# Autodesk Inventor assembly: Grundplatte_test
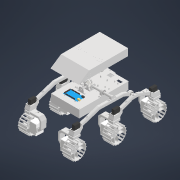
[picture p0: Inventor's stored thumbnail of the model, 180x180]
Saved by Autodesk Inventor 2021 (Build 250183000, 183)
## iProperties
Created: 2021-01-26
Part Number: Grundplatte_test
Document SubType Name: Assembly
Designer: Ctroi
Author: Ctroi
## Documents named in this file (39)
- E:\Projects\Rover\Grundplatte_test.iam
- E:\Projects\Rover\Grundplatte_hinten.ipt
- E:\Projects\Rover\Grundplatte_vorne.ipt
- E:\Projects\Rover\ArduinoMega.ipt
- E:\Projects\Rover\Kreuz_Halterung.ipt
- E:\Projects\Rover\Obenplatte_hinten.ipt
- E:\Projects\Rover\Obenplatte_vorne.ipt
- E:\Projects\Rover\Halterung_Differential_3.ipt
- E:\Projects\Rover\Halterung_Differential_Mitte.ipt
- E:\Projects\Rover\Halterung_Differential.ipt
- E:\Projects\Rover\Halterung_Differential_2.ipt
- E:\Projects\Rover\Kugellager.ipt
- E:\Projects\Rover\Kugellager_klein.ipt
- E:\Projects\Rover\Verbindung_Rocker_Body.ipt
- E:\Projects\Rover\Welle_Kugellager_Mitte.ipt
- E:\Projects\Rover\Rocker_hinten_rechts.ipt
- E:\Projects\Rover\Rocker_hinten.ipt
- E:\Projects\Rover\Rocker_vorne.ipt
- E:\Projects\Rover\Bogie.ipt
- E:\Projects\Rover\Boogie_Stange.ipt
- E:\Projects\Rover\Servohalterung_v2.ipt
- E:\Projects\Rover\Servo.ipt
- E:\Projects\Rover\Gegenstück_Welle_Diff.ipt
- E:\Projects\Rover\Zahnrad_innen.ipt
- E:\Projects\Rover\Übersetzungsbox_2.ipt
- E:\Projects\Rover\Zahnrad_außen.ipt
- E:\Projects\Rover\Motor_Servo_Welle_Test.ipt
- E:\Projects\Rover\Verbindung_Motor_Servo_v2.ipt
- E:\Projects\Rover\Motorhalterung_Klemme.ipt
- E:\Projects\Rover\Motorhalterung_v2.ipt
- E:\Projects\Rover\Steppermotor.ipt
- E:\Projects\Rover\Reifen_v2.ipt
- E:\Projects\Rover\Kegelrad.ipt
- E:\Projects\Rover\Relais.ipt
- E:\Projects\Rover\Kabelhalterung.ipt
- E:\Projects\Rover\Ebene3_vorne.ipt
- E:\Projects\Rover\Ebene3_mitte_vorne.ipt
- E:\Projects\Rover\Ebene3_hinten.ipt
- E:\Projects\Rover\Ebene3_verbindung.ipt
## Components (123 placed, 37 different names)
1. Relais:1 — Passend:208, Passend:209, Passend:210
2. Relais:2 — Passend:211, Passend:212, Passend:213
3. ArduinoMega:2 — Passend:228, Passend:229, Passend:230
4. Kabelhalterung:1 — Passend:234, Passend:235, Passend:236
5. Kabelhalterung:2 — Passend:237, Passend:238, Passend:239
6. Kabelhalterung:3 — Passend:231, Passend:232, Passend:233
7. Kabelhalterung:4 — Passend:240, Passend:241, Passend:242
8. Ebene3_vorne:1 — Passend:243, Passend:244, Passend:245, Passend:249, Passend:251
9. Ebene3_mitte_vorne:1 — Passend:246, Passend:247, Passend:248, Passend:250, Passend:252, Passend:253, Passend:254, Passend:255, Passend:256, Passend:257
10. Ebene3_hinten:1 — Passend:258, Passend:259, Passend:260
11. Ebene3_verbindung:1 — Passend:249, Passend:250, Passend:251
12. Ebene3_verbindung:2 — Passend:243, Passend:244, Passend:245, Passend:246, Passend:247, Passend:248
13. Ebene3_verbindung:3 — Passend:252, Passend:253, Passend:254
14. Ebene3_verbindung:4 — Passend:255, Passend:256, Passend:257, Passend:258, Passend:259, Passend:260
15. Grundplatte_hinten:1 — Passend:1, Passend:2, Passend:5, Passend:6, Passend:7, Passend:11, Passend:12, Passend:13, Passend:16, Passend:208, Passend:209, Passend:210, Passend:211, Passend:212, Passend:213
16. Grundplatte_vorne:1 — Passend:1, Passend:2, Passend:8, Passend:9, Passend:10, Passend:16, Passend:205, Passend:206, Passend:207
17. ArduinoMega:1 — Passend:205, Passend:206, Passend:207
18. Kreuz_Halterung:1 — Passend:5, Passend:6, Passend:7
19. Kegelrad2:1 — Passend:194, Passend:195
20. Kegelrad2:2 — Passend:196, Passend:197
21. Kegelrad2:3 — Passend:203, Passend:204
22. Gegenstück_Welle_Diff:1 — Passend:96, Passend:97
23. Welle_Kugellager_Mitte:1 — Passend:48, Passend:49, Passend:96, Passend:97, Passend:201, Passend:203, Passend:204
24. Obenplatte_vorne:1 — Passend:8, Passend:9, Passend:10, Passend:214, Passend:215, Passend:216, Passend:217, Passend:220, Passend:223, Passend:224, Passend:226, Passend:227, Passend:228, Passend:229, Passend:230, Passend:237, Passend:238, Passend:239, Passend:240, Passend:241, Passend:242
25. Halterung_Differential_3:1 — Passend:38, Passend:39, Passend:225, Passend:226, Passend:227
26. Halterung_Differential_3:2 — Passend:32, Passend:33, Passend:222, Passend:223, Passend:224
27. Obenplatte_hinten:1 — Passend:11, Passend:12, Passend:13, Passend:218, Passend:219, Passend:221, Passend:222, Passend:225, Passend:231, Passend:232, Passend:233, Passend:234, Passend:235, Passend:236
28. Halterung_Differential_Mitte:1 — Passend:42, Passend:43, Passend:214, Passend:215, Passend:216
29. Halterung_Differential:1 — Passend:36, Passend:37, Passend:199, Passend:200, Passend:217, Passend:218, Passend:219
30. Halterung_Differential:2 — Passend:34, Passend:35, Passend:198, Passend:220, Passend:221
31. Halterung_Differential_2:1 — Passend:198, Passend:199, Passend:200, Passend:201, Passend:202
32. Kugellager:1 — Passend:48, Passend:49, Passend:202
33. Kugellager:2 — Passend:32, Passend:33, Passend:47
34. Kugellager:3 — Passend:34, Passend:35, Passend:44
35. Kugellager:4 — Passend:36, Passend:37, Passend:45
36. Kugellager:5 — Passend:38, Passend:39, Passend:46
37. Kugellager_klein:1 — Passend:42, Passend:43
38. Reifen_v2:6 — Einfügen:3
39. Reifen_v2:5 — Einfügen:4
40. Reifen_v2:4 — Einfügen:5
41. Steppermotor:6 — Passend:191, Passend:192, Passend:193, Einfügen:5
42. Steppermotor:5 — Passend:188, Passend:189, Passend:190, Einfügen:4
43. Steppermotor:4 — Passend:185, Passend:186, Passend:187, Einfügen:3
44. Motorhalterung_v2:3 — Fluchtend:41, Fluchtend:42, Passend:170, Passend:185, Passend:186, Passend:187
45. Motorhalterung_v2:2 — Fluchtend:43, Fluchtend:44, Passend:171, Passend:188, Passend:189, Passend:190
46. Motorhalterung_v2:1 — Fluchtend:45, Fluchtend:46, Passend:172, Passend:191, Passend:192, Passend:193
47. Motorhalterung_Klemme:3 — Fluchtend:33, Fluchtend:34, Passend:166, Fluchtend:45, Fluchtend:46, Passend:172
48. Motorhalterung_Klemme:2 — Fluchtend:31, Fluchtend:32, Passend:165, Fluchtend:43, Fluchtend:44, Passend:171
49. Motorhalterung_Klemme:1 — Fluchtend:29, Fluchtend:30, Passend:164, Fluchtend:41, Fluchtend:42, Passend:170
50. Verbindung_Motor_Servo_v2:6 — Passend:158, Passend:159, Fluchtend:29, Fluchtend:30, Passend:164
51. Verbindung_Motor_Servo_v2:5 — Passend:162, Passend:163, Fluchtend:33, Fluchtend:34, Passend:166
52. Verbindung_Motor_Servo_v2:4 — Passend:160, Passend:161, Fluchtend:31, Fluchtend:32, Passend:165
53. Motor_Servo_Welle_Test:6 — Passend:150, Passend:151, Passend:158, Passend:159
54. Motor_Servo_Welle_Test:5 — Passend:148, Passend:149, Passend:162, Passend:163
55. Motor_Servo_Welle_Test:4 — Passend:146, Passend:147, Passend:160, Passend:161
56. Zahnrad_außen:6 — Passend:136, Passend:137
57. Zahnrad_außen:5 — Passend:138, Passend:139
58. Zahnrad_außen:4 — Passend:134, Passend:135
59. Kugellager:14 — Passend:122, Passend:123, Passend:148, Passend:149
60. Kugellager:13 — Passend:124, Passend:125, Passend:146, Passend:147
61. Kugellager:10 — Passend:126, Passend:127, Passend:150, Passend:151
62. Übersetzungsbox_2:6 — Fluchtend:25, Fluchtend:26, Passend:114, Passend:124, Passend:125
63. Übersetzungsbox_2:3 — Fluchtend:27, Fluchtend:28, Passend:115, Passend:122, Passend:123
64. Übersetzungsbox_2:2 — Fluchtend:19, Fluchtend:20, Passend:111, Passend:126, Passend:127
65. Zahnrad_innen:3 — Passend:102, Passend:103, Passend:136, Passend:137
66. Zahnrad_innen:2 — Passend:100, Passend:101, Passend:138, Passend:139
67. Zahnrad_innen:1 — Passend:98, Passend:99, Passend:134, Passend:135
68. Servo:3 — Passend:81, Passend:82, Passend:83, Passend:102, Passend:103
69. Servo:5 — Passend:93, Passend:94, Passend:95, Passend:100, Passend:101
70. Servo:2 — Passend:90, Passend:91, Passend:92, Passend:98, Passend:99
71. Servohalterung_v2:5 — Fluchtend:15, Fluchtend:16, Passend:77, Passend:90, Passend:91, Passend:92, Fluchtend:19, Fluchtend:20, Passend:111
72. Servohalterung_v2:3 — Fluchtend:13, Fluchtend:14, Passend:76, Passend:93, Passend:94, Passend:95, Fluchtend:25, Fluchtend:26, Passend:114
73. Servohalterung_v2:2 — Fluchtend:11, Fluchtend:12, Passend:75, Passend:81, Passend:82, Passend:83, Fluchtend:27, Fluchtend:28, Passend:115
74. Boogie_Stange:1 — Passend:64, Passend:65, Passend:68, Passend:69
75. Fahrwerk_bogie:2 — Passend:68, Passend:69, Fluchtend:13, Fluchtend:14, Passend:76, Fluchtend:15, Fluchtend:16, Passend:77
76. Fahrwerk_rocker_vorne:1 — Fluchtend:1, Fluchtend:2, Passend:62, Fluchtend:11, Fluchtend:12, Passend:75
77. Kugellager:7 — Passend:54, Passend:55, Passend:64, Passend:65
78. Kugellager:6 — Passend:52, Passend:53
79. Fahrwerk_rocker_hinten:1 — Passend:50, Passend:51, Passend:52, Passend:53, Passend:54, Passend:55, Fluchtend:1, Fluchtend:2, Passend:62
80. Verbindung_Rocker_Body:1 — Passend:44, Passend:47, Passend:50, Passend:51, Passend:194, Passend:195
81. Reifen_v2:3 — Einfügen:2
82. Reifen_v2:2 — Einfügen:1
83. Reifen_v2:1 — Einfügen:6
84. Steppermotor:3 — Passend:182, Passend:183, Passend:184, Einfügen:6
85. Steppermotor:2 — Passend:179, Passend:180, Passend:181, Einfügen:2
86. Steppermotor:1 — Passend:176, Passend:177, Passend:178, Einfügen:1
87. Motorhalterung_v2:6 — Fluchtend:51, Fluchtend:52, Passend:175, Passend:182, Passend:183, Passend:184
88. Motorhalterung_v2:5 — Fluchtend:49, Fluchtend:50, Passend:174, Passend:179, Passend:180, Passend:181
89. Motorhalterung_v2:4 — Fluchtend:47, Fluchtend:48, Passend:173, Passend:176, Passend:177, Passend:178
90. Motorhalterung_Klemme:4 — Fluchtend:35, Fluchtend:36, Passend:167, Fluchtend:47, Fluchtend:48, Passend:173
91. Motorhalterung_Klemme:5 — Fluchtend:37, Fluchtend:38, Passend:168, Fluchtend:49, Fluchtend:50, Passend:174
92. Motorhalterung_Klemme:6 — Fluchtend:39, Fluchtend:40, Passend:169, Fluchtend:51, Fluchtend:52, Passend:175
93. Verbindung_Motor_Servo_v2:3 — Passend:152, Passend:153, Fluchtend:35, Fluchtend:36, Passend:167
94. Verbindung_Motor_Servo_v2:2 — Passend:156, Passend:157, Fluchtend:39, Fluchtend:40, Passend:169
95. Verbindung_Motor_Servo_v2:1 — Passend:154, Passend:155, Fluchtend:37, Fluchtend:38, Passend:168
96. Motor_Servo_Welle_Test:3 — Passend:144, Passend:145, Passend:156, Passend:157
97. Motor_Servo_Welle_Test:2 — Passend:140, Passend:141, Passend:152, Passend:153
98. Motor_Servo_Welle_Test:1 — Passend:142, Passend:143, Passend:154, Passend:155
99. Zahnrad_außen:3 — Passend:132, Passend:133
100. Zahnrad_außen:2 — Passend:130, Passend:131
101. Zahnrad_außen:1 — Passend:128, Passend:129
102. Kugellager:15 — Passend:120, Passend:121, Passend:140, Passend:141
103. Kugellager:12 — Passend:118, Passend:119, Passend:142, Passend:143
104. Kugellager:11 — Passend:116, Passend:117, Passend:144, Passend:145
105. Übersetzungsbox_2:5 — Fluchtend:21, Fluchtend:22, Passend:112, Passend:118, Passend:119
106. Übersetzungsbox_2:4 — Fluchtend:23, Fluchtend:24, Passend:113, Passend:120, Passend:121
107. Übersetzungsbox_2:1 — Fluchtend:17, Fluchtend:18, Passend:110, Passend:116, Passend:117
108. Zahnrad_innen:6 — Passend:108, Passend:109, Passend:132, Passend:133
109. Zahnrad_innen:5 — Passend:106, Passend:107, Passend:130, Passend:131
110. Zahnrad_innen:4 — Passend:104, Passend:105, Passend:128, Passend:129
111. Servo:4 — Passend:78, Passend:79, Passend:80, Passend:108, Passend:109
112. Servo:6 — Passend:84, Passend:85, Passend:86, Passend:106, Passend:107
113. Servo:1 — Passend:87, Passend:88, Passend:89, Passend:104, Passend:105
114. Servohalterung_v2:6 — Fluchtend:5, Fluchtend:6, Passend:72, Passend:87, Passend:88, Passend:89, Fluchtend:17, Fluchtend:18, Passend:110
115. Servohalterung_v2:4 — Fluchtend:7, Fluchtend:8, Passend:73, Passend:84, Passend:85, Passend:86, Fluchtend:21, Fluchtend:22, Passend:112
116. Servohalterung_v2:1 — Fluchtend:9, Fluchtend:10, Passend:74, Passend:78, Passend:79, Passend:80, Fluchtend:23, Fluchtend:24, Passend:113
117. Boogie_Stange:2 — Passend:66, Passend:67, Passend:70, Passend:71
118. Fahrwerk_bogie:1 — Passend:70, Passend:71, Fluchtend:5, Fluchtend:6, Passend:72, Fluchtend:7, Fluchtend:8, Passend:73
119. Kugellager:9 — Passend:60, Passend:61
120. Kugellager:8 — Passend:58, Passend:59, Passend:66, Passend:67
121. Fahrwerk_rocker_hinten:2 — Passend:56, Passend:57, Passend:58, Passend:59, Passend:60, Passend:61, Fluchtend:3, Fluchtend:4, Passend:63
122. Fahrwerk_rocker_vorne:2 — Fluchtend:3, Fluchtend:4, Passend:63, Fluchtend:9, Fluchtend:10, Passend:74
123. Verbindung_Rocker_Body:2 — Passend:45, Passend:46, Passend:56, Passend:57, Passend:196, Passend:197
## Relationships (297: Mate 239, Flush 52, Insert 6)
- Passend:1 [Mate]: Grundplatte_hinten:1 ↔ Grundplatte_vorne:1
- Passend:2 [Mate]: Grundplatte_hinten:1 ↔ Grundplatte_vorne:1
- Passend:5 [Mate]: Grundplatte_hinten:1 ↔ Kreuz_Halterung:1
- Passend:6 [Mate]: Grundplatte_hinten:1 ↔ Kreuz_Halterung:1
- Passend:7 [Mate]: Grundplatte_hinten:1 ↔ Kreuz_Halterung:1
- Passend:8 [Mate]: Grundplatte_vorne:1 ↔ Obenplatte_vorne:1
- Passend:9 [Mate]: Grundplatte_vorne:1 ↔ Obenplatte_vorne:1
- Passend:10 [Mate]: Grundplatte_vorne:1 ↔ Obenplatte_vorne:1
- Passend:11 [Mate]: Grundplatte_hinten:1 ↔ Obenplatte_hinten:1
- Passend:12 [Mate]: Grundplatte_hinten:1 ↔ Obenplatte_hinten:1
- Passend:13 [Mate]: Grundplatte_hinten:1 ↔ Obenplatte_hinten:1
- Passend:16 [Mate]: Grundplatte_hinten:1 ↔ Grundplatte_vorne:1
- Passend:32 [Mate]: Halterung_Differential_3:2 ↔ Kugellager:2
- Passend:33 [Mate]: Halterung_Differential_3:2 ↔ Kugellager:2
- Passend:34 [Mate]: Halterung_Differential:2 ↔ Kugellager:3
- Passend:35 [Mate]: Halterung_Differential:2 ↔ Kugellager:3
- Passend:36 [Mate]: Halterung_Differential:1 ↔ Kugellager:4
- Passend:37 [Mate]: Halterung_Differential:1 ↔ Kugellager:4
- Passend:38 [Mate]: Halterung_Differential_3:1 ↔ Kugellager:5
- Passend:39 [Mate]: Halterung_Differential_3:1 ↔ Kugellager:5
- Passend:42 [Mate]: Halterung_Differential_Mitte:1 ↔ Kugellager_klein:1
- Passend:43 [Mate]: Halterung_Differential_Mitte:1 ↔ Kugellager_klein:1
- Passend:44 [Mate]: Kugellager:3 ↔ Verbindung_Rocker_Body:1
- Passend:45 [Mate]: Kugellager:4 ↔ Verbindung_Rocker_Body:2
- Passend:46 [Mate]: Kugellager:5 ↔ Verbindung_Rocker_Body:2
- Passend:47 [Mate]: Kugellager:2 ↔ Verbindung_Rocker_Body:1
- Passend:48 [Mate]: Welle_Kugellager_Mitte:1 ↔ Kugellager:1
- Passend:49 [Mate]: Welle_Kugellager_Mitte:1 ↔ Kugellager:1
- Passend:50 [Mate]: Fahrwerk_rocker_hinten:1 ↔ Verbindung_Rocker_Body:1
- Passend:51 [Mate]: Fahrwerk_rocker_hinten:1 ↔ Verbindung_Rocker_Body:1
- Passend:52 [Mate]: Kugellager:6 ↔ Fahrwerk_rocker_hinten:1
- Passend:53 [Mate]: Kugellager:6 ↔ Fahrwerk_rocker_hinten:1
- Passend:54 [Mate]: Kugellager:7 ↔ Fahrwerk_rocker_hinten:1
- Passend:55 [Mate]: Kugellager:7 ↔ Fahrwerk_rocker_hinten:1
- Passend:56 [Mate]: Fahrwerk_rocker_hinten:2 ↔ Verbindung_Rocker_Body:2
- Passend:57 [Mate]: Fahrwerk_rocker_hinten:2 ↔ Verbindung_Rocker_Body:2
- Passend:58 [Mate]: Kugellager:8 ↔ Fahrwerk_rocker_hinten:2
- Passend:59 [Mate]: Kugellager:8 ↔ Fahrwerk_rocker_hinten:2
- Passend:60 [Mate]: Kugellager:9 ↔ Fahrwerk_rocker_hinten:2
- Passend:61 [Mate]: Kugellager:9 ↔ Fahrwerk_rocker_hinten:2
- Fluchtend:1 [Flush]: Fahrwerk_rocker_vorne:1 ↔ Fahrwerk_rocker_hinten:1
- Fluchtend:2 [Flush]: Fahrwerk_rocker_vorne:1 ↔ Fahrwerk_rocker_hinten:1
- Passend:62 [Mate]: Fahrwerk_rocker_vorne:1 ↔ Fahrwerk_rocker_hinten:1
- Fluchtend:3 [Flush]: Fahrwerk_rocker_hinten:2 ↔ Fahrwerk_rocker_vorne:2
- Fluchtend:4 [Flush]: Fahrwerk_rocker_hinten:2 ↔ Fahrwerk_rocker_vorne:2
- Passend:63 [Mate]: Fahrwerk_rocker_hinten:2 ↔ Fahrwerk_rocker_vorne:2
- Passend:64 [Mate]: Boogie_Stange:1 ↔ Kugellager:7
- Passend:65 [Mate]: Boogie_Stange:1 ↔ Kugellager:7
- Passend:66 [Mate]: Boogie_Stange:2 ↔ Kugellager:8
- Passend:67 [Mate]: Boogie_Stange:2 ↔ Kugellager:8
- Passend:68 [Mate]: Boogie_Stange:1 ↔ Fahrwerk_bogie:2
- Passend:69 [Mate]: Boogie_Stange:1 ↔ Fahrwerk_bogie:2
- Passend:70 [Mate]: Boogie_Stange:2 ↔ Fahrwerk_bogie:1
- Passend:71 [Mate]: Boogie_Stange:2 ↔ Fahrwerk_bogie:1
- Fluchtend:5 [Flush]: Servohalterung_v2:6 ↔ Fahrwerk_bogie:1
- Fluchtend:6 [Flush]: Servohalterung_v2:6 ↔ Fahrwerk_bogie:1
- Passend:72 [Mate]: Servohalterung_v2:6 ↔ Fahrwerk_bogie:1
- Fluchtend:7 [Flush]: Servohalterung_v2:4 ↔ Fahrwerk_bogie:1
- Fluchtend:8 [Flush]: Servohalterung_v2:4 ↔ Fahrwerk_bogie:1
- Passend:73 [Mate]: Servohalterung_v2:4 ↔ Fahrwerk_bogie:1
- Fluchtend:9 [Flush]: Servohalterung_v2:1 ↔ Fahrwerk_rocker_vorne:2
- Fluchtend:10 [Flush]: Servohalterung_v2:1 ↔ Fahrwerk_rocker_vorne:2
- Passend:74 [Mate]: Servohalterung_v2:1 ↔ Fahrwerk_rocker_vorne:2
- Fluchtend:11 [Flush]: Servohalterung_v2:2 ↔ Fahrwerk_rocker_vorne:1
- Fluchtend:12 [Flush]: Servohalterung_v2:2 ↔ Fahrwerk_rocker_vorne:1
- Passend:75 [Mate]: Servohalterung_v2:2 ↔ Fahrwerk_rocker_vorne:1
- Fluchtend:13 [Flush]: Servohalterung_v2:3 ↔ Fahrwerk_bogie:2
- Fluchtend:14 [Flush]: Servohalterung_v2:3 ↔ Fahrwerk_bogie:2
- Passend:76 [Mate]: Servohalterung_v2:3 ↔ Fahrwerk_bogie:2
- Fluchtend:15 [Flush]: Servohalterung_v2:5 ↔ Fahrwerk_bogie:2
- Fluchtend:16 [Flush]: Servohalterung_v2:5 ↔ Fahrwerk_bogie:2
- Passend:77 [Mate]: Servohalterung_v2:5 ↔ Fahrwerk_bogie:2
- Passend:78 [Mate]: Servo:4 ↔ Servohalterung_v2:1
- Passend:79 [Mate]: Servo:4 ↔ Servohalterung_v2:1
- Passend:80 [Mate]: Servo:4 ↔ Servohalterung_v2:1
- Passend:81 [Mate]: Servo:3 ↔ Servohalterung_v2:2
- Passend:82 [Mate]: Servo:3 ↔ Servohalterung_v2:2
- Passend:83 [Mate]: Servo:3 ↔ Servohalterung_v2:2
- Passend:84 [Mate]: Servo:6 ↔ Servohalterung_v2:4
- Passend:85 [Mate]: Servo:6 ↔ Servohalterung_v2:4
- Passend:86 [Mate]: Servo:6 ↔ Servohalterung_v2:4
- Passend:87 [Mate]: Servo:1 ↔ Servohalterung_v2:6
- Passend:88 [Mate]: Servo:1 ↔ Servohalterung_v2:6
- Passend:89 [Mate]: Servo:1 ↔ Servohalterung_v2:6
- Passend:90 [Mate]: Servo:2 ↔ Servohalterung_v2:5
- Passend:91 [Mate]: Servo:2 ↔ Servohalterung_v2:5
- Passend:92 [Mate]: Servo:2 ↔ Servohalterung_v2:5
- Passend:93 [Mate]: Servo:5 ↔ Servohalterung_v2:3
- Passend:94 [Mate]: Servo:5 ↔ Servohalterung_v2:3
- Passend:95 [Mate]: Servo:5 ↔ Servohalterung_v2:3
- Passend:96 [Mate]: Gegenstück_Welle_Diff:1 ↔ Welle_Kugellager_Mitte:1
- Passend:97 [Mate]: Gegenstück_Welle_Diff:1 ↔ Welle_Kugellager_Mitte:1
- Passend:98 [Mate]: Zahnrad_innen:1 ↔ Servo:2
- Passend:99 [Mate]: Zahnrad_innen:1 ↔ Servo:2
- Passend:100 [Mate]: Zahnrad_innen:2 ↔ Servo:5
- Passend:101 [Mate]: Zahnrad_innen:2 ↔ Servo:5
- Passend:102 [Mate]: Zahnrad_innen:3 ↔ Servo:3
- Passend:103 [Mate]: Zahnrad_innen:3 ↔ Servo:3
- Passend:104 [Mate]: Zahnrad_innen:4 ↔ Servo:1
- Passend:105 [Mate]: Zahnrad_innen:4 ↔ Servo:1
- Passend:106 [Mate]: Zahnrad_innen:5 ↔ Servo:6
- Passend:107 [Mate]: Zahnrad_innen:5 ↔ Servo:6
- Passend:108 [Mate]: Zahnrad_innen:6 ↔ Servo:4
- Passend:109 [Mate]: Zahnrad_innen:6 ↔ Servo:4
- Fluchtend:17 [Flush]: Übersetzungsbox_2:1 ↔ Servohalterung_v2:6
- Fluchtend:18 [Flush]: Übersetzungsbox_2:1 ↔ Servohalterung_v2:6
- Passend:110 [Mate]: Übersetzungsbox_2:1 ↔ Servohalterung_v2:6
- Fluchtend:19 [Flush]: Übersetzungsbox_2:2 ↔ Servohalterung_v2:5
- Fluchtend:20 [Flush]: Übersetzungsbox_2:2 ↔ Servohalterung_v2:5
- Passend:111 [Mate]: Übersetzungsbox_2:2 ↔ Servohalterung_v2:5
- Fluchtend:21 [Flush]: Übersetzungsbox_2:5 ↔ Servohalterung_v2:4
- Fluchtend:22 [Flush]: Übersetzungsbox_2:5 ↔ Servohalterung_v2:4
- Passend:112 [Mate]: Übersetzungsbox_2:5 ↔ Servohalterung_v2:4
- Fluchtend:23 [Flush]: Übersetzungsbox_2:4 ↔ Servohalterung_v2:1
- Fluchtend:24 [Flush]: Übersetzungsbox_2:4 ↔ Servohalterung_v2:1
- Passend:113 [Mate]: Übersetzungsbox_2:4 ↔ Servohalterung_v2:1
- Fluchtend:25 [Flush]: Übersetzungsbox_2:6 ↔ Servohalterung_v2:3
- Fluchtend:26 [Flush]: Übersetzungsbox_2:6 ↔ Servohalterung_v2:3
- Passend:114 [Mate]: Übersetzungsbox_2:6 ↔ Servohalterung_v2:3
- Fluchtend:27 [Flush]: Übersetzungsbox_2:3 ↔ Servohalterung_v2:2
- Fluchtend:28 [Flush]: Übersetzungsbox_2:3 ↔ Servohalterung_v2:2
- Passend:115 [Mate]: Übersetzungsbox_2:3 ↔ Servohalterung_v2:2
- Passend:116 [Mate]: Kugellager:11 ↔ Übersetzungsbox_2:1
- Passend:117 [Mate]: Kugellager:11 ↔ Übersetzungsbox_2:1
- Passend:118 [Mate]: Kugellager:12 ↔ Übersetzungsbox_2:5
- Passend:119 [Mate]: Kugellager:12 ↔ Übersetzungsbox_2:5
- Passend:120 [Mate]: Kugellager:15 ↔ Übersetzungsbox_2:4
- Passend:121 [Mate]: Kugellager:15 ↔ Übersetzungsbox_2:4
- Passend:122 [Mate]: Kugellager:14 ↔ Übersetzungsbox_2:3
- Passend:123 [Mate]: Kugellager:14 ↔ Übersetzungsbox_2:3
- Passend:124 [Mate]: Kugellager:13 ↔ Übersetzungsbox_2:6
- Passend:125 [Mate]: Kugellager:13 ↔ Übersetzungsbox_2:6
- Passend:126 [Mate]: Kugellager:10 ↔ Übersetzungsbox_2:2
- Passend:127 [Mate]: Kugellager:10 ↔ Übersetzungsbox_2:2
- Passend:128 [Mate]: Zahnrad_außen:1 ↔ Zahnrad_innen:4
- Passend:129 [Mate]: Zahnrad_außen:1 ↔ Zahnrad_innen:4
- Passend:130 [Mate]: Zahnrad_außen:2 ↔ Zahnrad_innen:5
- Passend:131 [Mate]: Zahnrad_außen:2 ↔ Zahnrad_innen:5
- Passend:132 [Mate]: Zahnrad_außen:3 ↔ Zahnrad_innen:6
- Passend:133 [Mate]: Zahnrad_außen:3 ↔ Zahnrad_innen:6
- Passend:134 [Mate]: Zahnrad_außen:4 ↔ Zahnrad_innen:1
- Passend:135 [Mate]: Zahnrad_außen:4 ↔ Zahnrad_innen:1
- Passend:136 [Mate]: Zahnrad_außen:6 ↔ Zahnrad_innen:3
- Passend:137 [Mate]: Zahnrad_außen:6 ↔ Zahnrad_innen:3
- Passend:138 [Mate]: Zahnrad_außen:5 ↔ Zahnrad_innen:2
- Passend:139 [Mate]: Zahnrad_außen:5 ↔ Zahnrad_innen:2
- Passend:140 [Mate]: Motor_Servo_Welle_Test:2 ↔ Kugellager:15
- Passend:141 [Mate]: Motor_Servo_Welle_Test:2 ↔ Kugellager:15
- Passend:142 [Mate]: Motor_Servo_Welle_Test:1 ↔ Kugellager:12
- Passend:143 [Mate]: Motor_Servo_Welle_Test:1 ↔ Kugellager:12
- Passend:144 [Mate]: Motor_Servo_Welle_Test:3 ↔ Kugellager:11
- Passend:145 [Mate]: Motor_Servo_Welle_Test:3 ↔ Kugellager:11
- Passend:146 [Mate]: Motor_Servo_Welle_Test:4 ↔ Kugellager:13
- Passend:147 [Mate]: Motor_Servo_Welle_Test:4 ↔ Kugellager:13
- Passend:148 [Mate]: Motor_Servo_Welle_Test:5 ↔ Kugellager:14
- Passend:149 [Mate]: Motor_Servo_Welle_Test:5 ↔ Kugellager:14
- Passend:150 [Mate]: Motor_Servo_Welle_Test:6 ↔ Kugellager:10
- Passend:151 [Mate]: Motor_Servo_Welle_Test:6 ↔ Kugellager:10
- Passend:152 [Mate]: Verbindung_Motor_Servo_v2:3 ↔ Motor_Servo_Welle_Test:2
- Passend:153 [Mate]: Verbindung_Motor_Servo_v2:3 ↔ Motor_Servo_Welle_Test:2
- Passend:154 [Mate]: Verbindung_Motor_Servo_v2:1 ↔ Motor_Servo_Welle_Test:1
- Passend:155 [Mate]: Verbindung_Motor_Servo_v2:1 ↔ Motor_Servo_Welle_Test:1
- Passend:156 [Mate]: Verbindung_Motor_Servo_v2:2 ↔ Motor_Servo_Welle_Test:3
- Passend:157 [Mate]: Verbindung_Motor_Servo_v2:2 ↔ Motor_Servo_Welle_Test:3
- Passend:158 [Mate]: Verbindung_Motor_Servo_v2:6 ↔ Motor_Servo_Welle_Test:6
- Passend:159 [Mate]: Verbindung_Motor_Servo_v2:6 ↔ Motor_Servo_Welle_Test:6
- Passend:160 [Mate]: Verbindung_Motor_Servo_v2:4 ↔ Motor_Servo_Welle_Test:4
- Passend:161 [Mate]: Verbindung_Motor_Servo_v2:4 ↔ Motor_Servo_Welle_Test:4
- Passend:162 [Mate]: Verbindung_Motor_Servo_v2:5 ↔ Motor_Servo_Welle_Test:5
- Passend:163 [Mate]: Verbindung_Motor_Servo_v2:5 ↔ Motor_Servo_Welle_Test:5
- Fluchtend:29 [Flush]: Motorhalterung_Klemme:1 ↔ Verbindung_Motor_Servo_v2:6
- Fluchtend:30 [Flush]: Motorhalterung_Klemme:1 ↔ Verbindung_Motor_Servo_v2:6
- Passend:164 [Mate]: Motorhalterung_Klemme:1 ↔ Verbindung_Motor_Servo_v2:6
- Fluchtend:31 [Flush]: Motorhalterung_Klemme:2 ↔ Verbindung_Motor_Servo_v2:4
- Fluchtend:32 [Flush]: Motorhalterung_Klemme:2 ↔ Verbindung_Motor_Servo_v2:4
- Passend:165 [Mate]: Motorhalterung_Klemme:2 ↔ Verbindung_Motor_Servo_v2:4
- Fluchtend:33 [Flush]: Motorhalterung_Klemme:3 ↔ Verbindung_Motor_Servo_v2:5
- Fluchtend:34 [Flush]: Motorhalterung_Klemme:3 ↔ Verbindung_Motor_Servo_v2:5
- Passend:166 [Mate]: Motorhalterung_Klemme:3 ↔ Verbindung_Motor_Servo_v2:5
- Fluchtend:35 [Flush]: Motorhalterung_Klemme:4 ↔ Verbindung_Motor_Servo_v2:3
- Fluchtend:36 [Flush]: Motorhalterung_Klemme:4 ↔ Verbindung_Motor_Servo_v2:3
- Passend:167 [Mate]: Motorhalterung_Klemme:4 ↔ Verbindung_Motor_Servo_v2:3
- Fluchtend:37 [Flush]: Motorhalterung_Klemme:5 ↔ Verbindung_Motor_Servo_v2:1
- Fluchtend:38 [Flush]: Motorhalterung_Klemme:5 ↔ Verbindung_Motor_Servo_v2:1
- Passend:168 [Mate]: Motorhalterung_Klemme:5 ↔ Verbindung_Motor_Servo_v2:1
- Fluchtend:39 [Flush]: Motorhalterung_Klemme:6 ↔ Verbindung_Motor_Servo_v2:2
- Fluchtend:40 [Flush]: Motorhalterung_Klemme:6 ↔ Verbindung_Motor_Servo_v2:2
- Passend:169 [Mate]: Motorhalterung_Klemme:6 ↔ Verbindung_Motor_Servo_v2:2
- Fluchtend:41 [Flush]: Motorhalterung_v2:3 ↔ Motorhalterung_Klemme:1
- Fluchtend:42 [Flush]: Motorhalterung_v2:3 ↔ Motorhalterung_Klemme:1
- Passend:170 [Mate]: Motorhalterung_v2:3 ↔ Motorhalterung_Klemme:1
- Fluchtend:43 [Flush]: Motorhalterung_v2:2 ↔ Motorhalterung_Klemme:2
- Fluchtend:44 [Flush]: Motorhalterung_v2:2 ↔ Motorhalterung_Klemme:2
- Passend:171 [Mate]: Motorhalterung_v2:2 ↔ Motorhalterung_Klemme:2
- Fluchtend:45 [Flush]: Motorhalterung_v2:1 ↔ Motorhalterung_Klemme:3
- Fluchtend:46 [Flush]: Motorhalterung_v2:1 ↔ Motorhalterung_Klemme:3
- Passend:172 [Mate]: Motorhalterung_v2:1 ↔ Motorhalterung_Klemme:3
- Fluchtend:47 [Flush]: Motorhalterung_v2:4 ↔ Motorhalterung_Klemme:4
- Fluchtend:48 [Flush]: Motorhalterung_v2:4 ↔ Motorhalterung_Klemme:4
- Passend:173 [Mate]: Motorhalterung_v2:4 ↔ Motorhalterung_Klemme:4
- Fluchtend:49 [Flush]: Motorhalterung_v2:5 ↔ Motorhalterung_Klemme:5
- Fluchtend:50 [Flush]: Motorhalterung_v2:5 ↔ Motorhalterung_Klemme:5
- Passend:174 [Mate]: Motorhalterung_v2:5 ↔ Motorhalterung_Klemme:5
- Fluchtend:51 [Flush]: Motorhalterung_v2:6 ↔ Motorhalterung_Klemme:6
- Fluchtend:52 [Flush]: Motorhalterung_v2:6 ↔ Motorhalterung_Klemme:6
- Passend:175 [Mate]: Motorhalterung_v2:6 ↔ Motorhalterung_Klemme:6
- Passend:176 [Mate]: Steppermotor:1 ↔ Motorhalterung_v2:4
- Passend:177 [Mate]: Steppermotor:1 ↔ Motorhalterung_v2:4
- Passend:178 [Mate]: Steppermotor:1 ↔ Motorhalterung_v2:4
- Passend:179 [Mate]: Steppermotor:2 ↔ Motorhalterung_v2:5
- Passend:180 [Mate]: Steppermotor:2 ↔ Motorhalterung_v2:5
- Passend:181 [Mate]: Steppermotor:2 ↔ Motorhalterung_v2:5
- Passend:182 [Mate]: Steppermotor:3 ↔ Motorhalterung_v2:6
- Passend:183 [Mate]: Steppermotor:3 ↔ Motorhalterung_v2:6
- Passend:184 [Mate]: Steppermotor:3 ↔ Motorhalterung_v2:6
- Passend:185 [Mate]: Steppermotor:4 ↔ Motorhalterung_v2:3
- Passend:186 [Mate]: Steppermotor:4 ↔ Motorhalterung_v2:3
- Passend:187 [Mate]: Steppermotor:4 ↔ Motorhalterung_v2:3
- Passend:188 [Mate]: Steppermotor:5 ↔ Motorhalterung_v2:2
- Passend:189 [Mate]: Steppermotor:5 ↔ Motorhalterung_v2:2
- Passend:190 [Mate]: Steppermotor:5 ↔ Motorhalterung_v2:2
- Passend:191 [Mate]: Steppermotor:6 ↔ Motorhalterung_v2:1
- Passend:192 [Mate]: Steppermotor:6 ↔ Motorhalterung_v2:1
- Passend:193 [Mate]: Steppermotor:6 ↔ Motorhalterung_v2:1
- Einfügen:1 [Insert] (-15 mm): Reifen_v2:2 ↔ Steppermotor:1
- Einfügen:2 [Insert] (-15 mm): Reifen_v2:3 ↔ Steppermotor:2
- Einfügen:3 [Insert] (-15 mm): Reifen_v2:6 ↔ Steppermotor:4
- Einfügen:4 [Insert] (-15 mm): Reifen_v2:5 ↔ Steppermotor:5
- Einfügen:5 [Insert] (-15 mm): Reifen_v2:4 ↔ Steppermotor:6
- Passend:194 [Mate]: Kegelrad2:1 ↔ Verbindung_Rocker_Body:1
- Passend:195 [Mate]: Kegelrad2:1 ↔ Verbindung_Rocker_Body:1
- Passend:196 [Mate]: Kegelrad2:2 ↔ Verbindung_Rocker_Body:2
- Passend:197 [Mate]: Kegelrad2:2 ↔ Verbindung_Rocker_Body:2
- Passend:198 [Mate]: Halterung_Differential:2 ↔ Halterung_Differential_2:1
- Passend:199 [Mate]: Halterung_Differential:1 ↔ Halterung_Differential_2:1
- Passend:200 [Mate]: Halterung_Differential:1 ↔ Halterung_Differential_2:1
- Passend:201 [Mate]: Welle_Kugellager_Mitte:1 ↔ Halterung_Differential_2:1
- Passend:202 [Mate]: Halterung_Differential_2:1 ↔ Kugellager:1
- Passend:203 [Mate]: Kegelrad2:3 ↔ Welle_Kugellager_Mitte:1
- Passend:204 [Mate]: Kegelrad2:3 ↔ Welle_Kugellager_Mitte:1
- Einfügen:6 [Insert] (-15 mm): Reifen_v2:1 ↔ Steppermotor:3
- Passend:205 [Mate]: Grundplatte_vorne:1 ↔ ArduinoMega:1
- Passend:206 [Mate]: Grundplatte_vorne:1 ↔ ArduinoMega:1
- Passend:207 [Mate]: Grundplatte_vorne:1 ↔ ArduinoMega:1
- Passend:208 [Mate]: Relais:1 ↔ Grundplatte_hinten:1
- Passend:209 [Mate]: Relais:1 ↔ Grundplatte_hinten:1
- Passend:210 [Mate]: Relais:1 ↔ Grundplatte_hinten:1
- Passend:211 [Mate]: Relais:2 ↔ Grundplatte_hinten:1
- Passend:212 [Mate]: Relais:2 ↔ Grundplatte_hinten:1
- Passend:213 [Mate]: Relais:2 ↔ Grundplatte_hinten:1
- Passend:214 [Mate]: Obenplatte_vorne:1 ↔ Halterung_Differential_Mitte:1
- Passend:215 [Mate]: Obenplatte_vorne:1 ↔ Halterung_Differential_Mitte:1
- Passend:216 [Mate]: Obenplatte_vorne:1 ↔ Halterung_Differential_Mitte:1
- Passend:217 [Mate]: Obenplatte_vorne:1 ↔ Halterung_Differential:1
- Passend:218 [Mate]: Obenplatte_hinten:1 ↔ Halterung_Differential:1
- Passend:219 [Mate]: Obenplatte_hinten:1 ↔ Halterung_Differential:1
- Passend:220 [Mate]: Obenplatte_vorne:1 ↔ Halterung_Differential:2
- Passend:221 [Mate]: Obenplatte_hinten:1 ↔ Halterung_Differential:2
- Passend:222 [Mate]: Halterung_Differential_3:2 ↔ Obenplatte_hinten:1
- Passend:223 [Mate]: Obenplatte_vorne:1 ↔ Halterung_Differential_3:2
- Passend:224 [Mate]: Obenplatte_vorne:1 ↔ Halterung_Differential_3:2
- Passend:225 [Mate]: Halterung_Differential_3:1 ↔ Obenplatte_hinten:1
- Passend:226 [Mate]: Obenplatte_vorne:1 ↔ Halterung_Differential_3:1
- Passend:227 [Mate]: Obenplatte_vorne:1 ↔ Halterung_Differential_3:1
- Passend:228 [Mate]: ArduinoMega:2 ↔ Obenplatte_vorne:1
- Passend:229 [Mate]: ArduinoMega:2 ↔ Obenplatte_vorne:1
- Passend:230 [Mate]: ArduinoMega:2 ↔ Obenplatte_vorne:1
- Passend:231 [Mate]: Kabelhalterung:3 ↔ Obenplatte_hinten:1
- Passend:232 [Mate]: Kabelhalterung:3 ↔ Obenplatte_hinten:1
- Passend:233 [Mate]: Kabelhalterung:3 ↔ Obenplatte_hinten:1
- Passend:234 [Mate]: Kabelhalterung:1 ↔ Obenplatte_hinten:1
- Passend:235 [Mate]: Kabelhalterung:1 ↔ Obenplatte_hinten:1
- Passend:236 [Mate]: Kabelhalterung:1 ↔ Obenplatte_hinten:1
- Passend:237 [Mate]: Kabelhalterung:2 ↔ Obenplatte_vorne:1
- Passend:238 [Mate]: Kabelhalterung:2 ↔ Obenplatte_vorne:1
- Passend:239 [Mate]: Kabelhalterung:2 ↔ Obenplatte_vorne:1
- Passend:240 [Mate]: Kabelhalterung:4 ↔ Obenplatte_vorne:1
- Passend:241 [Mate]: Kabelhalterung:4 ↔ Obenplatte_vorne:1
- Passend:242 [Mate]: Kabelhalterung:4 ↔ Obenplatte_vorne:1
- Passend:243 [Mate]: Ebene3_vorne:1 ↔ Ebene3_verbindung:2
- Passend:244 [Mate]: Ebene3_vorne:1 ↔ Ebene3_verbindung:2
- Passend:245 [Mate]: Ebene3_vorne:1 ↔ Ebene3_verbindung:2
- Passend:246 [Mate]: Ebene3_mitte_vorne:1 ↔ Ebene3_verbindung:2
- Passend:247 [Mate]: Ebene3_mitte_vorne:1 ↔ Ebene3_verbindung:2
- Passend:248 [Mate]: Ebene3_mitte_vorne:1 ↔ Ebene3_verbindung:2
- Passend:249 [Mate]: Ebene3_vorne:1 ↔ Ebene3_verbindung:1
- Passend:250 [Mate]: Ebene3_mitte_vorne:1 ↔ Ebene3_verbindung:1
- Passend:251 [Mate]: Ebene3_vorne:1 ↔ Ebene3_verbindung:1
- Passend:252 [Mate]: Ebene3_mitte_vorne:1 ↔ Ebene3_verbindung:3
- Passend:253 [Mate]: Ebene3_mitte_vorne:1 ↔ Ebene3_verbindung:3
- Passend:254 [Mate]: Ebene3_mitte_vorne:1 ↔ Ebene3_verbindung:3
- Passend:255 [Mate]: Ebene3_mitte_vorne:1 ↔ Ebene3_verbindung:4
- Passend:256 [Mate]: Ebene3_mitte_vorne:1 ↔ Ebene3_verbindung:4
- Passend:257 [Mate]: Ebene3_mitte_vorne:1 ↔ Ebene3_verbindung:4
- Passend:258 [Mate]: Ebene3_hinten:1 ↔ Ebene3_verbindung:4
- Passend:259 [Mate]: Ebene3_hinten:1 ↔ Ebene3_verbindung:4
- Passend:260 [Mate]: Ebene3_hinten:1 ↔ Ebene3_verbindung:4
